# Autodesk Inventor assembly: Microlab_Electrical_CAD
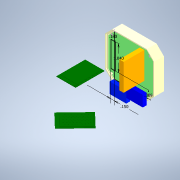
[picture p0: Inventor's stored thumbnail of the model, 180x180]
Saved by Autodesk Inventor 2022 (Build 260153000, 153)
## iProperties
Created: 2021-09-30
Part Number: Microlab_Electrical_CAD
Document SubType Name: Assembly
Designer: iss
Author: iss
## Documents named in this file (11)
- C:\Users\r8003\Downloads\Microlab_Next_CAD.iam
- C:\Users\r8003\Downloads\TPA6021A4EVM.ipt
- C:\Users\r8003\Downloads\AD9833Teyleten.ipt
- C:\Users\r8003\Downloads\MicroLab_Center_Shell.ipt
- C:\Users\r8003\Downloads\APS3008S-R.ipt
- C:\Users\r8003\Downloads\C329-SPI.ipt
- C:\Users\r8003\Downloads\MicroLab_Rear_Cover.ipt
- C:\Users\r8003\Downloads\MicroLab_Front_Cover.ipt
- C:\Users\r8003\Downloads\MicroLab_PCB_002.ipt
- C:\Users\r8003\Downloads\TPA2016.ipt
- C:\Users\r8003\Downloads\TPA2016_MIR.ipt
## Components (12 placed, 10 different names)
1. TPA6021A4EVM:1
2. AD9833Teyleten:1 — Mate:23, Mate:24, Mate:25, Mate:26, Mate:27, Mate:28, Mate:29, Flush:11
3. MicroLab_Center_Shell:1 — Flush:2, Mate:5, Mate:6, Mate:13, Mate:14, Mate:19, Mate:21, Angle:1, Flush:5, Mate:33, Mate:34, Mate:35, Mate:36
4. AD9833Teyleten:2 — Mate:28, Mate:29, Mate:30
5. APS3008S-R:1 — Mate:34, Mate:35
6. APS3008S-R:2 — Mate:33, Mate:36
7. C329-SPI:1 — Mate:16, Mate:17, Mate:18, Flush:6, Mate:26, Flush:7, Mate:32, Flush:9
8. MicroLab_Rear_Cover:1 — Mate:1, Flush:1, Mate:5, Mate:6, Mate:11, Mate:12, Mate:15, Flush:12, Flush:13, Flush:15, Flush:16
9. MicroLab_Front_Cover:1
10. MicroLab_PCB_002:1 — Mate:1, Flush:3, Mate:11, Mate:12, Flush:4, Mate:16, Mate:17, Mate:20, Flush:8
11. TPA2016:1 — Mate:19, Mate:20, Mate:22, Mate:23, Mate:24, Mate:30, Mate:31, Mate:32, Flush:10, Mate:37, Flush:14
12. TPA2016_MIR:1 — Mate:38, Mate:39, Flush:17, Mate:40, Flush:18
## Relationships (54: Mate 34, Flush 18, Angle 1, Symmetry 1)
- Mate:1: MicroLab_Rear_Cover:1 ↔ MicroLab_PCB_002:1
- Flush:1: MicroLab_Rear_Cover:1
- Flush:2: MicroLab_Center_Shell:1
- Mate:4
- Mate:5: MicroLab_Center_Shell:1 ↔ MicroLab_Rear_Cover:1
- Mate:6: MicroLab_Center_Shell:1 ↔ MicroLab_Rear_Cover:1
- Flush:3 (-17.018 mm): MicroLab_PCB_002:1
- Mate:11: MicroLab_Rear_Cover:1 ↔ MicroLab_PCB_002:1
- Mate:12: MicroLab_Rear_Cover:1 ↔ MicroLab_PCB_002:1
- Mate:13: MicroLab_Center_Shell:1
- Mate:14: MicroLab_Center_Shell:1
- Mate:15: MicroLab_Rear_Cover:1
- Flush:4 (-17.018 mm): MicroLab_PCB_002:1
- Mate:16 (3.429 mm): C329-SPI:1 ↔ MicroLab_PCB_002:1
- Mate:17: C329-SPI:1 ↔ MicroLab_PCB_002:1
- Mate:18: C329-SPI:1
- Mate:19: MicroLab_Center_Shell:1 ↔ TPA2016:1
- Mate:20 (7.588 mm): MicroLab_PCB_002:1 ↔ TPA2016:1
- Mate:21: MicroLab_Center_Shell:1
- Angle:1 (0 deg): MicroLab_Center_Shell:1
- Mate:22 (7.8486 mm): TPA2016:1
- Flush:5: MicroLab_Center_Shell:1
- Mate:23: AD9833Teyleten:1 ↔ TPA2016:1
- Mate:24: AD9833Teyleten:1 ↔ TPA2016:1
- Flush:6 (4 mm): C329-SPI:1
- Mate:25: AD9833Teyleten:1
- Mate:26: AD9833Teyleten:1 ↔ C329-SPI:1
- Flush:7: C329-SPI:1
- Mate:27: AD9833Teyleten:1
- Mate:28: AD9833Teyleten:1 ↔ AD9833Teyleten:2
- Mate:29: AD9833Teyleten:1 ↔ AD9833Teyleten:2
- Mate:30: AD9833Teyleten:2 ↔ TPA2016:1
- Flush:8 (4 mm): MicroLab_PCB_002:1
- Mate:31: TPA2016:1
- Mate:32 (4 mm): C329-SPI:1 ↔ TPA2016:1
- Flush:9: C329-SPI:1
- Flush:10: TPA2016:1
- Mate:33: MicroLab_Center_Shell:1 ↔ APS3008S-R:2
- Mate:34: MicroLab_Center_Shell:1 ↔ APS3008S-R:1
- Mate:35: MicroLab_Center_Shell:1 ↔ APS3008S-R:1
- Mate:36: MicroLab_Center_Shell:1 ↔ APS3008S-R:2
- Flush:11 (7 mm): AD9833Teyleten:1
- Mate:37: TPA2016:1
- Flush:12: MicroLab_Rear_Cover:1
- Flush:13: MicroLab_Rear_Cover:1
- Flush:14: TPA2016:1
- Flush:15: MicroLab_Rear_Cover:1
- Flush:16: MicroLab_Rear_Cover:1
- Symmetry:1
- Mate:38 (7.8486 mm): TPA2016_MIR:1
- Mate:39: TPA2016_MIR:1
- Flush:17: TPA2016_MIR:1
- Mate:40: TPA2016_MIR:1
- Flush:18: TPA2016_MIR:1
